# Autodesk Inventor assembly: NewScrewDrive
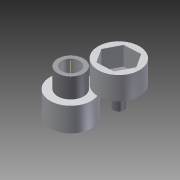
[picture p0: Inventor's stored thumbnail of the model, 180x180]
Saved by Autodesk Inventor 2012 (Build 160160000, 160)
## iProperties
Created: 2011-10-19
Part Number: NewScrewDrive
Document SubType Name: Assembly
Designer: KuttaA
Author: KuttaA
## Documents named in this file (3)
- C:\Users\KuttaA\Dropbox\Hexapod Research\Leg Design\Other Parts\NewScrewDrive.iam
- C:\Users\KuttaA\Dropbox\Hexapod Research\Leg Design\Other Parts\MotorToGear.ipt
- C:\Users\KuttaA\Dropbox\Hexapod Research\Leg Design\Other Parts\GearToScrew.ipt
## Components (2 placed, 2 different names)
1. MotorToGear:1 — Mate:3, Rotation:1, Angle:2, Mate:4, Mate:1
2. GearToScrew:1 — Rotation:1, Angle:2, Mate:1
## Relationships (5: Mate 3, RelateRotation 1, Angle 1)
- Mate:3: MotorToGear:1
- Rotation:1 [RelateRotation] (0.5 ul): MotorToGear:1 ↔ GearToScrew:1
- Angle:2 (180 deg): MotorToGear:1 ↔ GearToScrew:1
- Mate:4: MotorToGear:1
- Mate:1: MotorToGear:1 ↔ GearToScrew:1
